# Autodesk Inventor assembly: ServoHousingTest
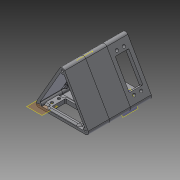
[picture p0: Inventor's stored thumbnail of the model, 180x180]
Saved by Autodesk Inventor 2014 SP1 (Build 180222100, 222)
## iProperties
Created: 2014-11-03
Part Number: ServoHousingTest
Document SubType Name: Assembly
Designer: rawrdong
Author: rawrdong
## Documents named in this file (2)
- C:\Users\rawrdong\Documents\GitHub\FlippityFlappity\CAD_HW\ServoHousingTest.iam
- C:\Users\rawrdong\Documents\GitHub\FlippityFlappity\CAD_HW\ServoHousing.ipt
## Components (3 placed, 1 different names)
1. ServoHousing:1 — Mate:1, Mate:2, Mate:3
2. ServoHousing:2 — Mate:1, Mate:2, Mate:3, Mate:4, Mate:5, Mate:6
3. ServoHousing:3 — Mate:4, Mate:5, Mate:6
## Relationships (6: Mate 6)
- Mate:1: ServoHousing:1 ↔ ServoHousing:2
- Mate:2: ServoHousing:1 ↔ ServoHousing:2
- Mate:3: ServoHousing:1 ↔ ServoHousing:2
- Mate:4: ServoHousing:2 ↔ ServoHousing:3
- Mate:5: ServoHousing:2 ↔ ServoHousing:3
- Mate:6: ServoHousing:2 ↔ ServoHousing:3
